# Autodesk Inventor assembly: 조립품1
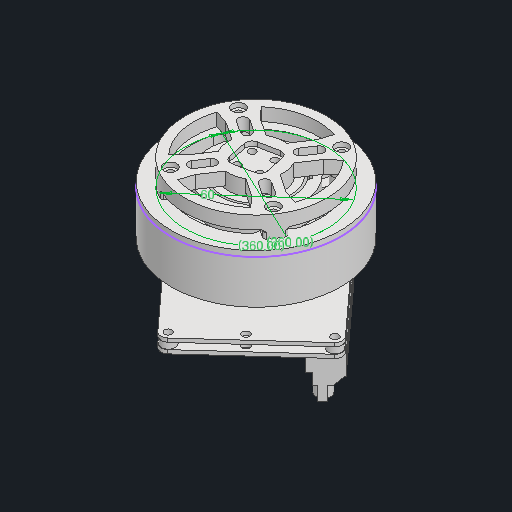
[picture p0: Inventor's stored thumbnail of the model, 512x512]
Saved by Autodesk Inventor 2025.1 (Build 291241020, 241B)
## iProperties
Created: 2025-07-23
Part Number: 조립품1
Document SubType Name: Assembly
Designer: acalo
Author: acalo
## Documents named in this file (11)
- C:\Users\acalo\OneDrive\바탕 화면\Design\6010BLDC\조립품1.iam
- C:\Users\acalo\OneDrive\바탕 화면\Design\6010BLDC\Dummy_Stator.ipt
- C:\Users\acalo\OneDrive\바탕 화면\Design\6010BLDC\Shaft_A.ipt
- C:\Users\acalo\OneDrive\바탕 화면\Design\6010BLDC\ShaftLock_A.ipt
- C:\Users\acalo\OneDrive\바탕 화면\Design\6010BLDC\6804zz.ipt
- C:\Users\acalo\OneDrive\바탕 화면\Design\6010BLDC\Rotator_B.ipt
- C:\Users\acalo\OneDrive\바탕 화면\Design\6010BLDC\Rotator_A_8PP.ipt
- C:\Users\acalo\OneDrive\바탕 화면\Design\6010BLDC\Test_block.ipt
- C:\Users\acalo\OneDrive\바탕 화면\Design\6010BLDC\Driver.ipt
- C:\Users\acalo\OneDrive\바탕 화면\Design\6010BLDC\Test_Shaft.ipt
- C:\Users\acalo\OneDrive\바탕 화면\Design\6010BLDC\Test_ShaftB.ipt
## Components (10 placed, 10 different names)
1. Dummy_Stator:1 — 플러쉬:1, 메이트:1
2. Shaft_A:1 — 플러쉬:1, 메이트:1, 메이트:2, 메이트:3, 메이트:4, 메이트:23, 메이트:24, 메이트:25
3. ShaftLock_A:1 — 메이트:2, 메이트:3, 메이트:4, 메이트:5, 플러쉬:2
4. 6804zz:1 — 메이트:5, 플러쉬:2, 메이트:21, 메이트:22
5. Rotator_B:1 — 메이트:18, 메이트:19, 메이트:20, 메이트:21, 메이트:22, 메이트:29
6. Rotator_A_8PP:1 — 메이트:18, 메이트:19, 메이트:20, 메이트:26, 메이트:27, 메이트:28
7. Test_block:1 — 메이트:23, 메이트:24, 메이트:25
8. Driver:1 — 메이트:26
9. Test_Shaft:1 — 메이트:27, 메이트:30
10. Test_ShaftB:1 — 메이트:28, 메이트:29, 메이트:30
## Relationships (20: Mate 18, Flush 2)
- 플러쉬:1 [Flush] (2 mm): Dummy_Stator:1 ↔ Shaft_A:1
- 메이트:1 [Mate]: Dummy_Stator:1 ↔ Shaft_A:1
- 메이트:2 [Mate]: Shaft_A:1 ↔ ShaftLock_A:1
- 메이트:3 [Mate]: Shaft_A:1 ↔ ShaftLock_A:1
- 메이트:4 [Mate]: Shaft_A:1 ↔ ShaftLock_A:1
- 메이트:5 [Mate]: ShaftLock_A:1 ↔ 6804zz:1
- 플러쉬:2 [Flush]: ShaftLock_A:1 ↔ 6804zz:1
- 메이트:18 [Mate]: Rotator_B:1 ↔ Rotator_A_8PP:1
- 메이트:19 [Mate]: Rotator_B:1 ↔ Rotator_A_8PP:1
- 메이트:20 [Mate]: Rotator_B:1 ↔ Rotator_A_8PP:1
- 메이트:21 [Mate]: 6804zz:1 ↔ Rotator_B:1
- 메이트:22 [Mate]: 6804zz:1 ↔ Rotator_B:1
- 메이트:23 [Mate]: Shaft_A:1 ↔ Test_block:1
- 메이트:24 [Mate]: Shaft_A:1 ↔ Test_block:1
- 메이트:25 [Mate]: Shaft_A:1 ↔ Test_block:1
- 메이트:26 [Mate]: Rotator_A_8PP:1 ↔ Driver:1
- 메이트:27 [Mate]: Rotator_A_8PP:1 ↔ Test_Shaft:1
- 메이트:28 [Mate]: Rotator_A_8PP:1 ↔ Test_ShaftB:1
- 메이트:29 [Mate]: Rotator_B:1 ↔ Test_ShaftB:1
- 메이트:30 [Mate]: Test_Shaft:1 ↔ Test_ShaftB:1
